# Autodesk Inventor assembly: Robot
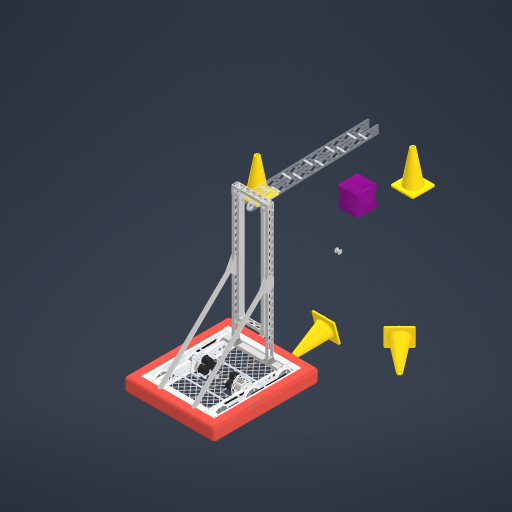
[picture p0: Inventor's stored thumbnail of the model, 512x512]
Saved by Autodesk Inventor 2023 (Build 270158000, 158)
## iProperties
Created: 2023-01-07
Part Number: Robot
Document SubType Name: Assembly
Designer: Blank Slate
Author: Blank Slate
## Documents named in this file (12)
- C:\Users\Terrence\Documents\FRC Long\Robot (1).iam
- C:\Users\Terrence\Documents\FRC Long\Parts\AM14U5 Long ToughBox Mini 6in HiGrip 6wD.iam
- C:\Users\Terrence\Documents\FRC Long\Parts\2+Stage+3+Motor+Evo+Shifter.iam
- C:\Users\Terrence\Documents\FRC Long\Parts\am-4258_15T NEO with 15T 32DP Pinion for EVO Gearboxes.ipt
- C:\Users\Terrence\Documents\FRC Long\Parts\bellypan.ipt
- C:\Users\Terrence\Documents\FRC Long\Bumper\Bumper.iam
- C:\Users\Terrence\Documents\FRC Long\Newvator\Elevator.iam
- C:\Users\Terrence\Downloads\60355K503_Ball Bearing (1).ipt
- C:\Users\Terrence\Documents\FRC Long\Tower\Tower.iam
- C:\Users\Terrence\Documents\FRC Long\Arm\Arm.iam
- C:\Users\Terrence\Documents\FRC Long\Cone.ipt
- C:\Users\Terrence\Documents\FRC Long\Cube.ipt
## Components (27 placed, 11 different names)
1. AM14U5 Long ToughBox Mini 6in HiGrip 6wD:1 [sub-assembly] — Insert:13, Insert:14, Insert:15, Insert:16, Insert:17, Insert:18, Flush:2, Mate:5, Mate:6, Mate:7, Flush:5, Mate:10
2. 2+Stage+3+Motor+Evo+Shifter:1 [sub-assembly] — Insert:1, Insert:2, Insert:3, Insert:4, Insert:5, Insert:6, Insert:15, Insert:16
3. am-4258_15T NEO with 15T 32DP Pinion for EVO Gearboxes:1 — Insert:1, Insert:2
4. am-4258_15T NEO with 15T 32DP Pinion for EVO Gearboxes:2 — Insert:3, Insert:4
5. am-4258_15T NEO with 15T 32DP Pinion for EVO Gearboxes:3 — Insert:5, Insert:6
6. 2+Stage+3+Motor+Evo+Shifter:2 [sub-assembly] — Insert:13, Insert:14
7. am-4258_15T NEO with 15T 32DP Pinion for EVO Gearboxes:4
8. am-4258_15T NEO with 15T 32DP Pinion for EVO Gearboxes:5
9. am-4258_15T NEO with 15T 32DP Pinion for EVO Gearboxes:6
10. bellypan:1 — Insert:17, Insert:18
11. Bumper:1 [sub-assembly] — Flush:2, Mate:5, Mate:6
12. Elevator:1 [sub-assembly] — Insert:19, Insert:22, Insert:26, Insert:27, Flush:4, Mate:9, Insert:28, Mate:14, Mate:15
13. 60355K503_Ball Bearing (1):1 — Insert:19, Insert:20
14. 60355K503_Ball Bearing (1):2 — Insert:20
15. 60355K503_Ball Bearing (1):3
16. 60355K503_Ball Bearing (1):4 — Insert:22
17. 60355K503_Ball Bearing (1):5 — Insert:27
18. 60355K503_Ball Bearing (1):6
19. 60355K503_Ball Bearing (1):7 — Insert:26
20. 60355K503_Ball Bearing (1):8
21. Tower:1 [sub-assembly] — Mate:7, Flush:4, Mate:9, Flush:5, Mate:10, Mate:14, Mate:15
22. Arm:1 [sub-assembly] — Insert:28
23. Cone:1
24. Cube:1
25. Cone:2
26. Cone:3
27. Cone:4
## Relationships (37: Insert 27, Mate 7, Flush 3)
- Insert:1: 2+Stage+3+Motor+Evo+Shifter:1 ↔ am-4258_15T NEO with 15T 32DP Pinion for EVO Gearboxes:1
- Insert:2: 2+Stage+3+Motor+Evo+Shifter:1 ↔ am-4258_15T NEO with 15T 32DP Pinion for EVO Gearboxes:1
- Insert:3: 2+Stage+3+Motor+Evo+Shifter:1 ↔ am-4258_15T NEO with 15T 32DP Pinion for EVO Gearboxes:2
- Insert:4: 2+Stage+3+Motor+Evo+Shifter:1 ↔ am-4258_15T NEO with 15T 32DP Pinion for EVO Gearboxes:2
- Insert:5: 2+Stage+3+Motor+Evo+Shifter:1 ↔ am-4258_15T NEO with 15T 32DP Pinion for EVO Gearboxes:3
- Insert:6: 2+Stage+3+Motor+Evo+Shifter:1 ↔ am-4258_15T NEO with 15T 32DP Pinion for EVO Gearboxes:3
- [Insert]: 2+Stage+3+Motor+Evo+Shifter:2 ↔ am-4258_15T NEO with 15T 32DP Pinion for EVO Gearboxes:4
- [Insert]: 2+Stage+3+Motor+Evo+Shifter:2 ↔ am-4258_15T NEO with 15T 32DP Pinion for EVO Gearboxes:4
- [Insert]: 2+Stage+3+Motor+Evo+Shifter:2 ↔ am-4258_15T NEO with 15T 32DP Pinion for EVO Gearboxes:5
- [Insert]: 2+Stage+3+Motor+Evo+Shifter:2 ↔ am-4258_15T NEO with 15T 32DP Pinion for EVO Gearboxes:5
- [Insert]: 2+Stage+3+Motor+Evo+Shifter:2 ↔ am-4258_15T NEO with 15T 32DP Pinion for EVO Gearboxes:6
- [Insert]: 2+Stage+3+Motor+Evo+Shifter:2 ↔ am-4258_15T NEO with 15T 32DP Pinion for EVO Gearboxes:6
- Insert:13: AM14U5 Long ToughBox Mini 6in HiGrip 6wD:1 ↔ 2+Stage+3+Motor+Evo+Shifter:2
- Insert:14: AM14U5 Long ToughBox Mini 6in HiGrip 6wD:1 ↔ 2+Stage+3+Motor+Evo+Shifter:2
- Insert:15: AM14U5 Long ToughBox Mini 6in HiGrip 6wD:1 ↔ 2+Stage+3+Motor+Evo+Shifter:1
- Insert:16: AM14U5 Long ToughBox Mini 6in HiGrip 6wD:1 ↔ 2+Stage+3+Motor+Evo+Shifter:1
- Insert:17: AM14U5 Long ToughBox Mini 6in HiGrip 6wD:1 ↔ bellypan:1
- Insert:18: AM14U5 Long ToughBox Mini 6in HiGrip 6wD:1 ↔ bellypan:1
- Flush:2: AM14U5 Long ToughBox Mini 6in HiGrip 6wD:1 ↔ Bumper:1
- Mate:5: AM14U5 Long ToughBox Mini 6in HiGrip 6wD:1 ↔ Bumper:1
- Mate:6: AM14U5 Long ToughBox Mini 6in HiGrip 6wD:1 ↔ Bumper:1
- Insert:19: Elevator:1 ↔ 60355K503_Ball Bearing (1):1
- Insert:20: 60355K503_Ball Bearing (1):1 ↔ 60355K503_Ball Bearing (1):2
- [Insert]: 60355K503_Ball Bearing (1):3 ↔ 60355K503_Ball Bearing (1):4
- Insert:22: Elevator:1 ↔ 60355K503_Ball Bearing (1):4
- [Insert]: 60355K503_Ball Bearing (1):5 ↔ 60355K503_Ball Bearing (1):6
- [Insert]: 60355K503_Ball Bearing (1):7 ↔ 60355K503_Ball Bearing (1):8
- Insert:26: Elevator:1 ↔ 60355K503_Ball Bearing (1):7
- Insert:27: Elevator:1 ↔ 60355K503_Ball Bearing (1):5
- Mate:7: AM14U5 Long ToughBox Mini 6in HiGrip 6wD:1 ↔ Tower:1
- Flush:4: Elevator:1 ↔ Tower:1
- Mate:9 (17.4625 mm): Elevator:1 ↔ Tower:1
- Flush:5: AM14U5 Long ToughBox Mini 6in HiGrip 6wD:1 ↔ Tower:1
- Mate:10 (25.4 mm): AM14U5 Long ToughBox Mini 6in HiGrip 6wD:1 ↔ Tower:1
- Insert:28: Elevator:1 ↔ Arm:1
- Mate:14: Elevator:1 ↔ Tower:1
- Mate:15: Elevator:1 ↔ Tower:1
## Named parameters: d6_d0 = 0 mm, d7_d1 = 0 mm, d8_d2 = 0 mm, d9_d3 = 0 mm, d10_d4 = 0 mm, d11_d5 = 0 mm, d167_d166 = 0 mm, d169_d166 = 0 mm, d171_d169_d166 = 0 mm
